# Autodesk Inventor assembly: OUTK_000_Assembly
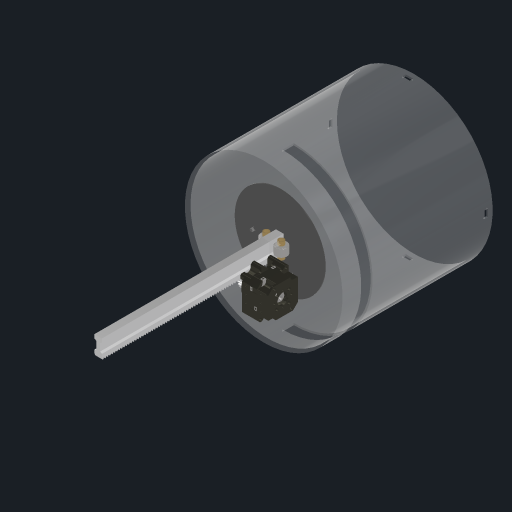
[picture p0: Inventor's stored thumbnail of the model, 512x512]
Saved by Autodesk Inventor 2024.2 (Build 282272000, 272)
## iProperties
Created: 2024-11-24
Part Number: OUTK_000_Assembly
Document SubType Name: Assembly
Designer: Bryan
Mass: 4347.94 g
Surface Area: 10314.1 cm^2
Volume: 2070.59 cm^3
Density: 2.09986 g/cm^3
Author: Bryan
## Documents named in this file (15)
- C:\Users\bobsb\OneDrive\Documents\GitHub\1622-2024-Casino-Clash-CAD-A-Thon\Outtake\OUTK_000_Assembly.iam
- C:\Users\bobsb\OneDrive\Documents\GitHub\1622-2024-Casino-Clash-CAD-A-Thon\Outtake\OUTK_002_ShotPlateNoReceptacle.ipt
- C:\Users\bobsb\OneDrive\Documents\GitHub\1622-2024-Casino-Clash-CAD-A-Thon\Outtake\OUTK_002_ShotPlateReceptacle.ipt
- C:\Users\bobsb\OneDrive\Documents\GitHub\1622-2024-Casino-Clash-CAD-A-Thon\Outtake\OUTK_001_ChipBucket.ipt
- C:\Users\bobsb\OneDrive\Documents\GitHub\1622-2024-Casino-Clash-CAD-A-Thon\Outtake\OUTK_004_PlanetaryShaft.ipt
- C:\Users\bobsb\OneDrive\Documents\GitHub\1622-2024-Casino-Clash-CAD-A-Thon\COTS Library\MAXPlanetary System\COTS_0.5inhexoutput_REV-21-2104.ipt
- C:\Users\bobsb\OneDrive\Documents\GitHub\1622-2024-Casino-Clash-CAD-A-Thon\COTS Library\MAXPlanetary System\COTS_5to1Stage_REV-21-2103.ipt
- C:\Users\bobsb\OneDrive\Documents\GitHub\1622-2024-Casino-Clash-CAD-A-Thon\COTS Library\MAXPlanetary System\COTS_InputStage_REV-21-2106.ipt
- C:\Users\bobsb\OneDrive\Documents\GitHub\1622-2024-Casino-Clash-CAD-A-Thon\COTS Library\MAXPlanetary System\COTS_NeoShaftAdapter_REV-21-2108.ipt
- C:\Users\bobsb\OneDrive\Documents\GitHub\1622-2024-Casino-Clash-CAD-A-Thon\COTS Library\Fasteners\Bolts\Button-Head\10-32\COTS_91255A265_Button Head Hex Drive Screw.ipt
- C:\Users\bobsb\OneDrive\Documents\GitHub\1622-2024-Casino-Clash-CAD-A-Thon\Outtake\OUTK_003_Metal Gear Rack, Modified.ipt
- C:\Users\bobsb\OneDrive\Documents\GitHub\1622-2024-Casino-Clash-CAD-A-Thon\Outtake\OUTK_006_OiliteBushing.ipt
- C:\Users\bobsb\OneDrive\Documents\GitHub\1622-2024-Casino-Clash-CAD-A-Thon\COTS Library\Motion\Wheels\Roller Wheels\COTS_6831K11_Shaft-Mount Flat Track Roller.ipt
- C:\Users\bobsb\OneDrive\Documents\GitHub\1622-2024-Casino-Clash-CAD-A-Thon\COTS Library\Motion\Gears\20DP gears\Aluminum\COTS_20DP20T_WCP-0701(1).ipt
- C:\Users\bobsb\OneDrive\Documents\GitHub\1622-2024-Casino-Clash-CAD-A-Thon\Outtake\OUTK_008_Plunger.ipt
## Components (20 placed, 14 different names)
1. OUTK_002_ShotPlateNoReceptacle:1 — Mate:4, Mate:5, Mate:41
2. OUTK_002_ShotPlateReceptacle:1 — Mate:3, Mate:4, Mate:5, Mate:41, Mate:42
3. OUTK_001_ChipBucket:1 — Mate:3, Mate:18, Mate:19, Mate:20, Mate:21, Mate:29, Angle:1, Tangent:5, Mate:42
4. OUTK_004_PlanetaryShaft:1 — Mate:8, Mate:9, Mate:10, Mate:40, Flush:3
5. COTS_0.5inhexoutput_REV-21-2104:1 — Mate:8, Mate:9, Mate:11, Mate:12, Flush:1, Mate:13, Mate:18, Mate:19
6. COTS_5to1Stage_REV-21-2103:1 — Mate:12, Flush:1, Mate:13, Flush:2, Mate:14, Mate:15, Mate:16, Mate:17, Mate:20
7. COTS_InputStage_REV-21-2106:1 — Flush:2, Mate:14, Mate:17
8. COTS_NeoShaftAdapter_REV-21-2108:1 — Mate:15, Mate:16
9. COTS_91255A265_Button Head Hex Drive Screw:1 — Mate:10, Mate:11
10. OUTK_003_Metal Gear Rack, Modified:1 — Mate:21, Tangent:1, Mate:29, Tangent:2, Mate:43, Mate:44, Mate:45, Mate:46, Mate:47, Mate:48, Mate:49
11. OUTK_006_OiliteBushing:1 — Mate:31, Mate:32
12. COTS_6831K11_Shaft-Mount Flat Track Roller:2 — Tangent:1, Tangent:4, Mate:35, Mate:36, Mate:37, Mate:38, Mate:44
13. COTS_6831K11_Shaft-Mount Flat Track Roller:3 — Tangent:2, Tangent:3, Mate:31, Mate:32, Mate:33, Mate:34, Tangent:5, Mate:43
14. OUTK_006_OiliteBushing:2 — Mate:33, Mate:34
15. OUTK_006_OiliteBushing:3 — Mate:35, Mate:36
16. OUTK_006_OiliteBushing:4 — Mate:37, Mate:38
17. COTS_20DP20T_WCP-0701(1):1 — Mate:40, Flush:3
18. OUTK_008_Plunger:1 — Mate:45, Mate:46, Mate:47, Mate:50, Mate:51
19. COTS_91255A265_Button Head Hex Drive Screw:2 — Mate:48, Mate:51
20. COTS_91255A265_Button Head Hex Drive Screw:3 — Mate:49, Mate:50
## Relationships (47: Mate 38, Tangent 5, Flush 3, Angle 1)
- Mate:3: OUTK_002_ShotPlateReceptacle:1 ↔ OUTK_001_ChipBucket:1
- Mate:4: OUTK_002_ShotPlateNoReceptacle:1 ↔ OUTK_002_ShotPlateReceptacle:1
- Mate:5: OUTK_002_ShotPlateNoReceptacle:1 ↔ OUTK_002_ShotPlateReceptacle:1
- Mate:8: OUTK_004_PlanetaryShaft:1 ↔ COTS_0.5inhexoutput_REV-21-2104:1
- Mate:9: OUTK_004_PlanetaryShaft:1 ↔ COTS_0.5inhexoutput_REV-21-2104:1
- Mate:10: OUTK_004_PlanetaryShaft:1 ↔ COTS_91255A265_Button Head Hex Drive Screw:1
- Mate:11: COTS_0.5inhexoutput_REV-21-2104:1 ↔ COTS_91255A265_Button Head Hex Drive Screw:1
- Mate:12: COTS_0.5inhexoutput_REV-21-2104:1 ↔ COTS_5to1Stage_REV-21-2103:1
- Flush:1: COTS_0.5inhexoutput_REV-21-2104:1 ↔ COTS_5to1Stage_REV-21-2103:1
- Mate:13: COTS_0.5inhexoutput_REV-21-2104:1 ↔ COTS_5to1Stage_REV-21-2103:1
- Flush:2: COTS_5to1Stage_REV-21-2103:1 ↔ COTS_InputStage_REV-21-2106:1
- Mate:14: COTS_5to1Stage_REV-21-2103:1 ↔ COTS_InputStage_REV-21-2106:1
- Mate:15: COTS_5to1Stage_REV-21-2103:1 ↔ COTS_NeoShaftAdapter_REV-21-2108:1
- Mate:16: COTS_5to1Stage_REV-21-2103:1 ↔ COTS_NeoShaftAdapter_REV-21-2108:1
- Mate:17: COTS_5to1Stage_REV-21-2103:1 ↔ COTS_InputStage_REV-21-2106:1
- Mate:18: OUTK_001_ChipBucket:1 ↔ COTS_0.5inhexoutput_REV-21-2104:1
- Mate:19: OUTK_001_ChipBucket:1 ↔ COTS_0.5inhexoutput_REV-21-2104:1
- Mate:20: OUTK_001_ChipBucket:1 ↔ COTS_5to1Stage_REV-21-2103:1
- Mate:21 (3.175 mm): OUTK_001_ChipBucket:1 ↔ OUTK_003_Metal Gear Rack, Modified:1
- Tangent:1: OUTK_003_Metal Gear Rack, Modified:1 ↔ COTS_6831K11_Shaft-Mount Flat Track Roller:2
- Mate:29 (3.175 mm): OUTK_001_ChipBucket:1 ↔ OUTK_003_Metal Gear Rack, Modified:1
- Tangent:2: OUTK_003_Metal Gear Rack, Modified:1 ↔ COTS_6831K11_Shaft-Mount Flat Track Roller:3
- Angle:1 (0 deg): OUTK_001_ChipBucket:1
- Tangent:3: COTS_6831K11_Shaft-Mount Flat Track Roller:3
- Tangent:4: COTS_6831K11_Shaft-Mount Flat Track Roller:2
- Mate:31: OUTK_006_OiliteBushing:1 ↔ COTS_6831K11_Shaft-Mount Flat Track Roller:3
- Mate:32: OUTK_006_OiliteBushing:1 ↔ COTS_6831K11_Shaft-Mount Flat Track Roller:3
- Mate:33: COTS_6831K11_Shaft-Mount Flat Track Roller:3 ↔ OUTK_006_OiliteBushing:2
- Mate:34: COTS_6831K11_Shaft-Mount Flat Track Roller:3 ↔ OUTK_006_OiliteBushing:2
- Mate:35: COTS_6831K11_Shaft-Mount Flat Track Roller:2 ↔ OUTK_006_OiliteBushing:3
- Mate:36: COTS_6831K11_Shaft-Mount Flat Track Roller:2 ↔ OUTK_006_OiliteBushing:3
- Mate:37: COTS_6831K11_Shaft-Mount Flat Track Roller:2 ↔ OUTK_006_OiliteBushing:4
- Mate:38: COTS_6831K11_Shaft-Mount Flat Track Roller:2 ↔ OUTK_006_OiliteBushing:4
- Tangent:5 (1.27 mm): OUTK_001_ChipBucket:1 ↔ COTS_6831K11_Shaft-Mount Flat Track Roller:3
- Mate:40: OUTK_004_PlanetaryShaft:1 ↔ COTS_20DP20T_WCP-0701(1):1
- Mate:41 (19.05 mm): OUTK_002_ShotPlateNoReceptacle:1 ↔ OUTK_002_ShotPlateReceptacle:1
- Mate:42: OUTK_002_ShotPlateReceptacle:1 ↔ OUTK_001_ChipBucket:1
- Flush:3: OUTK_004_PlanetaryShaft:1 ↔ COTS_20DP20T_WCP-0701(1):1
- Mate:43: OUTK_003_Metal Gear Rack, Modified:1 ↔ COTS_6831K11_Shaft-Mount Flat Track Roller:3
- Mate:44: OUTK_003_Metal Gear Rack, Modified:1 ↔ COTS_6831K11_Shaft-Mount Flat Track Roller:2
- Mate:45: OUTK_003_Metal Gear Rack, Modified:1 ↔ OUTK_008_Plunger:1
- Mate:46: OUTK_003_Metal Gear Rack, Modified:1 ↔ OUTK_008_Plunger:1
- Mate:47: OUTK_003_Metal Gear Rack, Modified:1 ↔ OUTK_008_Plunger:1
- Mate:48: OUTK_003_Metal Gear Rack, Modified:1 ↔ COTS_91255A265_Button Head Hex Drive Screw:2
- Mate:49: OUTK_003_Metal Gear Rack, Modified:1 ↔ COTS_91255A265_Button Head Hex Drive Screw:3
- Mate:50: OUTK_008_Plunger:1 ↔ COTS_91255A265_Button Head Hex Drive Screw:3
- Mate:51: OUTK_008_Plunger:1 ↔ COTS_91255A265_Button Head Hex Drive Screw:2
